# Autodesk Inventor assembly: terminal assembly
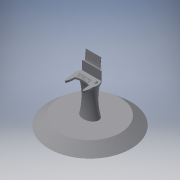
[picture p0: Inventor's stored thumbnail of the model, 180x180]
Saved by Autodesk Inventor 2017 (Build 210142000, 142)
## iProperties
Created: 2018-03-19
Part Number: terminal assembly
Document SubType Name: Assembly
Designer: Braxton
Author: Braxton
## Documents named in this file (5)
- D:\School\Game develpment\geoscape\done\terminal\assembly\terminal assembly without rails.iam
- D:\School\Game develpment\geoscape\done\terminal\terminal stand removed rails.ipt
- D:\School\Game develpment\geoscape\done\terminal\terminal use.ipt
- D:\School\Game develpment\geoscape\done\terminal\key board low tec.ipt
- D:\School\Game develpment\geoscape\done\terminal\terditional mouse.ipt
## Components (4 placed, 4 different names)
1. terminal stand removed rails:1 — Mate:6, Mate:8, Mate:10, Flush:1, Mate:15, Mate:16, Flush:2, Mate:17
2. terminal use:1 — Mate:8, Flush:2, Mate:17
3. key board low tec:1 — Mate:6, Flush:1, Mate:13, Mate:15
4. terditional mouse:1 — Mate:10, Mate:13, Mate:16
## Relationships (9: Mate 7, Flush 2)
- Mate:6: terminal stand removed rails:1 ↔ key board low tec:1
- Mate:8: terminal stand removed rails:1 ↔ terminal use:1
- Mate:10: terminal stand removed rails:1 ↔ terditional mouse:1
- Flush:1: terminal stand removed rails:1 ↔ key board low tec:1
- Mate:13: key board low tec:1 ↔ terditional mouse:1
- Mate:15: terminal stand removed rails:1 ↔ key board low tec:1
- Mate:16 (-2.1167 mm): terminal stand removed rails:1 ↔ terditional mouse:1
- Flush:2: terminal stand removed rails:1 ↔ terminal use:1
- Mate:17: terminal stand removed rails:1 ↔ terminal use:1
